# Autodesk Inventor assembly: Clippard 8-MC 3D PCB with silkscreen
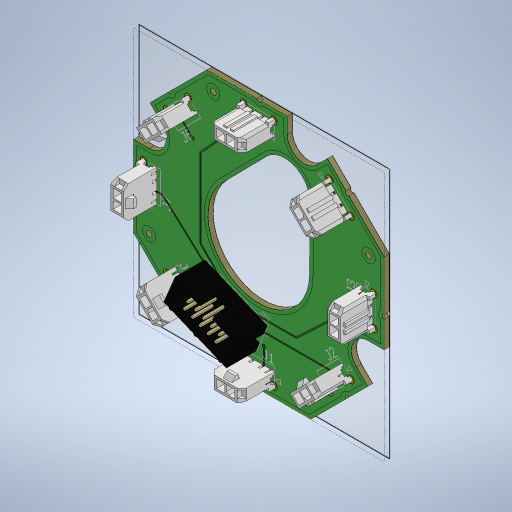
[picture p0: Inventor's stored thumbnail of the model, 512x512]
Saved by Autodesk Inventor 2024.2 (Build 282272000, 272)
## iProperties
Created: 2024-03-21
Part Number: Clippard 8-MC 3D PCB with silkscreen
Document SubType Name: Assembly
Designer: shann
Author: shann
## Documents named in this file (4)
- C:\Users\shann\Dropbox (NYU Langone Health)\OlfactometerEngineeringGroup (2)\Design\OlfaControl_Electronics\8-line Mixing Chamber\Clippard\Electronics\3D PCB\Clippard 8-MC_v01 with silkscreen.iam
- C:\Users\shann\Dropbox (NYU Langone Health)\OlfactometerEngineeringGroup (2)\Design\OlfaControl_Electronics\8-line Mixing Chamber\Clippard\Electronics\3D PCB\Clippard 8-MC_v01.iam
- C:\Users\shann\Dropbox (NYU Langone Health)\OlfactometerEngineeringGroup (2)\Design\OlfaControl_Electronics\8-line Mixing Chamber\Clippard\Electronics\3D PCB\3D PCB Components\silkscreen\Clippard 8-MC_v01 Top.ipt
- C:\Users\shann\Dropbox (NYU Langone Health)\OlfactometerEngineeringGroup (2)\Design\OlfaControl_Electronics\8-line Mixing Chamber\Clippard\Electronics\3D PCB\3D PCB Components\silkscreen\Clippard 8-MC_v01 Bottom.ipt
## Components (3 placed, 3 different names)
1. Clippard 8-MC_v01:1 [sub-assembly] — top silkscreen to PCB:1, top silkscreen to PCB:2, top silkscreen to PCB:3, btm silkscreen to PCB:1, btm silkscreen to PCB:2, btm silkscreen to PCB:3
2. Clippard 8-MC_v01 Top:1 — top silkscreen to PCB:1, top silkscreen to PCB:2, top silkscreen to PCB:3
3. Clippard 8-MC_v01 Bottom:1 — btm silkscreen to PCB:1, btm silkscreen to PCB:2, btm silkscreen to PCB:3
## Relationships (6: Flush 4, Mate 2)
- top silkscreen to PCB:1 [Flush]: Clippard 8-MC_v01:1 ↔ Clippard 8-MC_v01 Top:1
- top silkscreen to PCB:2 [Flush]: Clippard 8-MC_v01:1 ↔ Clippard 8-MC_v01 Top:1
- top silkscreen to PCB:3 [Mate]: Clippard 8-MC_v01:1 ↔ Clippard 8-MC_v01 Top:1
- btm silkscreen to PCB:1 [Flush]: Clippard 8-MC_v01:1 ↔ Clippard 8-MC_v01 Bottom:1
- btm silkscreen to PCB:2 [Flush]: Clippard 8-MC_v01:1 ↔ Clippard 8-MC_v01 Bottom:1
- btm silkscreen to PCB:3 [Mate]: Clippard 8-MC_v01:1 ↔ Clippard 8-MC_v01 Bottom:1
